# Autodesk Inventor assembly: Spider_Robot_Leg_Assembly_V1
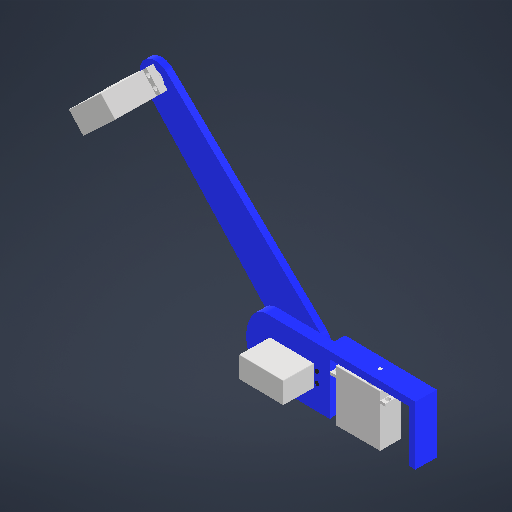
[picture p0: Inventor's stored thumbnail of the model, 512x512]
Saved by Autodesk Inventor 2026.2 (Build 302298010, 298A)
## iProperties
Created: 2026-07-24
Part Number: Spider_Robot_Leg_Assembly_V1
Document SubType Name: Assembly
Designer: Entity
Author: Entity
## Documents named in this file (5)
- C:\Users\Entity\OneDrive\Documents\Bells University of Technology Documents\Autodesk Inventor Projects\Spider_Robot_Leg_Assembly_V1.iam
- C:\Users\Entity\OneDrive\Documents\Bells University of Technology Documents\Autodesk Inventor Projects\Servo Part 1.ipt
- C:\Users\Entity\OneDrive\Documents\Bells University of Technology Documents\Autodesk Inventor Projects\Part1.ipt
- C:\Users\Entity\OneDrive\Documents\Bells University of Technology Documents\Autodesk Inventor Projects\Servo_Pin.ipt
- C:\Users\Entity\OneDrive\Documents\Bells University of Technology Documents\Autodesk Inventor Projects\Tibia.ipt
## Components (9 placed, 4 different names)
1. Part1:1 — Rotational:1, Insert:1, Insert:2, Insert:3, Insert:4
2. Servo Part 1:1 — Rotational:1
3. Servo Part 1:2 — Insert:5, Rotational:2
4. Servo_Pin:1 — Insert:3
5. Servo_Pin:2 — Insert:4
6. Servo_Pin:3 — Insert:2
7. Servo_Pin:4 — Insert:1, Insert:5
8. Tibia:1 — Rotational:2, Rotational:3
9. Servo Part 1:3 — Rotational:3
## Relationships (8: Insert 5, RevoluteJoint 3)
- Rotational:1 [RevoluteJoint]: Part1:1 ↔ Servo Part 1:1
- Insert:1: Part1:1 ↔ Servo_Pin:4
- Insert:2: Part1:1 ↔ Servo_Pin:3
- Insert:3: Part1:1 ↔ Servo_Pin:1
- Insert:4: Part1:1 ↔ Servo_Pin:2
- Insert:5: Servo Part 1:2 ↔ Servo_Pin:4
- Rotational:2 [RevoluteJoint]: Servo Part 1:2 ↔ Tibia:1
- Rotational:3 [RevoluteJoint]: Tibia:1 ↔ Servo Part 1:3
